# Autodesk Inventor assembly: součást
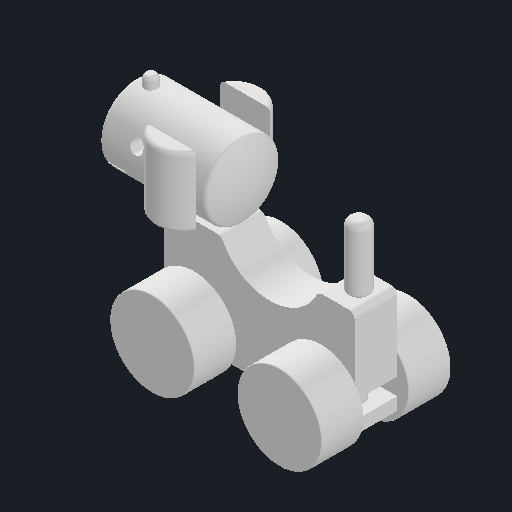
[picture p0: Inventor's stored thumbnail of the model, 512x512]
Saved by Autodesk Inventor 2025.1 (Build 291241000, 241)
## iProperties
Created: 2025-04-28
Part Number: součást
Document SubType Name: Assembly
Designer: Dominik Petříček
Author: Dominik Petříček
## Documents named in this file (5)
- D:\Škola\SŠ\4.ročník\Cad\Maturita\součást.iam
- D:\Škola\SŠ\4.ročník\Cad\Maturita\součást 1.ipt
- D:\Škola\SŠ\4.ročník\Cad\Maturita\součást 2.ipt
- D:\Škola\SŠ\4.ročník\Cad\Maturita\součást 3.ipt
- D:\Škola\SŠ\4.ročník\Cad\Maturita\součást 4.ipt
## Components (5 placed, 4 different names)
1. součást 1:1 — Rotační:1, Rotační:2, Rotační:3, Rotační:4
2. součást 2:1 — Rotační:2
3. součást 2:2 — Rotační:3
4. součást 3:1 — Rotační:4
5. součást 4:1 — Rotační:1
## Relationships (4: RevoluteJoint 4)
- Rotační:1 [RevoluteJoint]: součást 1:1 ↔ součást 4:1
- Rotační:2 [RevoluteJoint]: součást 1:1 ↔ součást 2:1
- Rotační:3 [RevoluteJoint]: součást 1:1 ↔ součást 2:2
- Rotační:4 [RevoluteJoint]: součást 1:1 ↔ součást 3:1
